# Autodesk Inventor assembly: SteelM-StarS
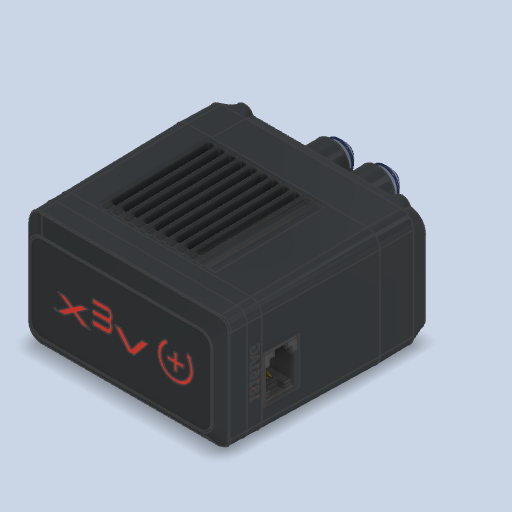
[picture p0: Inventor's stored thumbnail of the model, 512x512]
Saved by Autodesk Inventor 2026 (Build 300175000, 175)
## iProperties
Created: 2022-08-18
Part Number: SteelM-StarS
Document SubType Name: Assembly
Designer: avere
Author: ylu12
## Documents named in this file (4)
- C:\Users\avere\OneDrive\Documents\VEX-CAD\V5-CAD\drivetrain\Drivebay Right\SteelM-StarS.iam
- C:\Users\avere\OneDrive\Documents\VEX-CAD\V5-CAD\drivetrain\Drivebay Right\V5 Motor.ipt
- C:\Users\avere\OneDrive\Documents\VEX-CAD\VEX-CAD-Inventor\Structure\Hardware\Screw Steel - Star\SScrew Star Smooth .500.ipt
- C:\Users\avere\OneDrive\Documents\VEX-CAD\VEX-CAD-Inventor\Structure\Hardware\Screw Steel - Star.ipt
## Components (3 placed, 2 different names)
1. V5 Motor:1
2. SScrew Star Smooth .500:1
3. SScrew Star Smooth .500:2
## Named parameters: Thickness = 1.1938 mm
